# Autodesk Inventor assembly: Z Nut Bracket Assemby 1.0
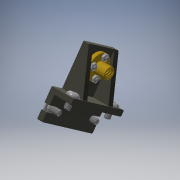
[picture p0: Inventor's stored thumbnail of the model, 180x180]
Saved by Autodesk Inventor 2016 (Build 200138000, 138)
## iProperties
Created: 2017-04-16
Part Number: Z Nut Bracket Assemby 1.0
Document SubType Name: Assembly
Designer: Scott
Author: Scott
## Documents named in this file (6)
- E:\Scott Projects\3D Printing\CoreXY\Z Nut Bracket Assemby 1.0.iam
- E:\Scott Projects\3D Printing\CoreXY\Z Nut Braket 1.0.ipt
- E:\Scott Projects\3D Printing\CoreXY\Trapezoidal lead screw Nut tr8x8-4.ipt
- C:\Users\Scott\Documents\Inventor\Content Center Files\R2016\en-US\ANSI B18.3.1M(1)\ANSI B18.3.1M - M3x0.5 x 12(2).ipt
- C:\Users\Scott\Documents\Inventor\Content Center Files\R2016\en-US\ISO 4032(2)\ISO 4032 - M3 - ISO.ipt
- C:\Users\Scott\Documents\Inventor\Content Center Files\R2016\en-US\ANSI B18.3.4M(1)\ANSI B18.3.4M - M5 x 0.8 x 10(2).ipt
## Components (14 placed, 5 different names)
1. Z Nut Braket 1.0:1 — Mate:1, Mate:2, Mate:3, Mate:8, Mate:9, Mate:10, Mate:11, Angle:1, Angle:2, Angle:3, Angle:4, Insert:5, Insert:6, Insert:7, Insert:8
2. Trapezoidal lead screw Nut tr8x8-4:1 — Mate:1, Mate:2, Mate:3, Mate:4, Mate:5, Mate:6, Mate:7, Insert:1, Insert:2, Insert:3, Insert:4
3. Broached Socket Head Cap Screw - Metric M3x0.5 x 12:1 — Mate:4, Mate:11
4. Broached Socket Head Cap Screw - Metric M3x0.5 x 12:2 — Mate:5, Mate:10
5. Broached Socket Head Cap Screw - Metric M3x0.5 x 12:3 — Mate:6, Mate:9
6. Broached Socket Head Cap Screw - Metric M3x0.5 x 12:4 — Mate:7, Mate:8
7. ISO 4032 M3:1 — Insert:2, Angle:4
8. ISO 4032 M3:2 — Insert:3, Angle:3
9. ISO 4032 M3:3 — Insert:4, Angle:1
10. ISO 4032 M3:4 — Insert:1, Angle:2
11. Broached Hexagon Socket Button Head Cap Screw - Metric M5 x 0.8 x 10:1 — Insert:7
12. Broached Hexagon Socket Button Head Cap Screw - Metric M5 x 0.8 x 10:2 — Insert:6
13. Broached Hexagon Socket Button Head Cap Screw - Metric M5 x 0.8 x 10:3 — Insert:5
14. Broached Hexagon Socket Button Head Cap Screw - Metric M5 x 0.8 x 10:4 — Insert:8
## Relationships (23: Mate 11, Insert 8, Angle 4)
- Mate:1: Z Nut Braket 1.0:1 ↔ Trapezoidal lead screw Nut tr8x8-4:1
- Mate:2: Z Nut Braket 1.0:1 ↔ Trapezoidal lead screw Nut tr8x8-4:1
- Mate:3 (22 mm): Z Nut Braket 1.0:1 ↔ Trapezoidal lead screw Nut tr8x8-4:1
- Mate:4: Trapezoidal lead screw Nut tr8x8-4:1 ↔ Broached Socket Head Cap Screw - Metric M3x0.5 x 12:1
- Mate:5: Trapezoidal lead screw Nut tr8x8-4:1 ↔ Broached Socket Head Cap Screw - Metric M3x0.5 x 12:2
- Mate:6: Trapezoidal lead screw Nut tr8x8-4:1 ↔ Broached Socket Head Cap Screw - Metric M3x0.5 x 12:3
- Mate:7: Trapezoidal lead screw Nut tr8x8-4:1 ↔ Broached Socket Head Cap Screw - Metric M3x0.5 x 12:4
- Mate:8: Z Nut Braket 1.0:1 ↔ Broached Socket Head Cap Screw - Metric M3x0.5 x 12:4
- Mate:9: Z Nut Braket 1.0:1 ↔ Broached Socket Head Cap Screw - Metric M3x0.5 x 12:3
- Mate:10: Z Nut Braket 1.0:1 ↔ Broached Socket Head Cap Screw - Metric M3x0.5 x 12:2
- Mate:11: Z Nut Braket 1.0:1 ↔ Broached Socket Head Cap Screw - Metric M3x0.5 x 12:1
- Insert:1: Trapezoidal lead screw Nut tr8x8-4:1 ↔ ISO 4032 M3:4
- Insert:2: Trapezoidal lead screw Nut tr8x8-4:1 ↔ ISO 4032 M3:1
- Insert:3: Trapezoidal lead screw Nut tr8x8-4:1 ↔ ISO 4032 M3:2
- Insert:4: Trapezoidal lead screw Nut tr8x8-4:1 ↔ ISO 4032 M3:3
- Angle:1 (0 deg): Z Nut Braket 1.0:1 ↔ ISO 4032 M3:3
- Angle:2 (0 deg): Z Nut Braket 1.0:1 ↔ ISO 4032 M3:4
- Angle:3 (0 deg): Z Nut Braket 1.0:1 ↔ ISO 4032 M3:2
- Angle:4 (0 deg): Z Nut Braket 1.0:1 ↔ ISO 4032 M3:1
- Insert:5: Z Nut Braket 1.0:1 ↔ Broached Hexagon Socket Button Head Cap Screw - Metric M5 x 0.8 x 10:3
- Insert:6: Z Nut Braket 1.0:1 ↔ Broached Hexagon Socket Button Head Cap Screw - Metric M5 x 0.8 x 10:2
- Insert:7: Z Nut Braket 1.0:1 ↔ Broached Hexagon Socket Button Head Cap Screw - Metric M5 x 0.8 x 10:1
- Insert:8: Z Nut Braket 1.0:1 ↔ Broached Hexagon Socket Button Head Cap Screw - Metric M5 x 0.8 x 10:4
